# Autodesk Inventor assembly: independent_wheel_pair
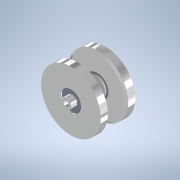
[picture p0: Inventor's stored thumbnail of the model, 180x180]
Saved by Autodesk Inventor 2020.3 (Build 243373000, 373)
## iProperties
Created: 2021-03-25
Part Number: independent_wheel_pair
Document SubType Name: Assembly
Designer: patry
Mass: 73.5609 g
Surface Area: 155.822 cm^2
Volume: 27.2448 cm^3
Density: 2.7 g/cm^3
Author: patry
## Documents named in this file (5)
- C:\Users\patry\Desktop\Konar staff\Ariadna2.1\ariadna_mechanika\Obszar roboczy\Naped\Zawieszenie_v3\independent_wheel_pair.iam
- C:\Users\patry\Desktop\Konar staff\Ariadna2.1\ariadna_mechanika\Obszar roboczy\Naped\Kola\single_wheel.iam
- C:\Users\patry\Desktop\Konar staff\Ariadna2.1\ariadna_mechanika\Obszar roboczy\Naped\Sruby\M5_nut_5mm.ipt
- C:\Users\patry\Desktop\Konar staff\Ariadna2.1\ariadna_mechanika\Obszar roboczy\Naped\Sruby\M5x35.ipt
- C:\Users\patry\Desktop\Konar staff\Ariadna2.1\ariadna_mechanika\Obszar roboczy\Naped\Sruby\M5_pad.ipt
## Components (7 placed, 4 different names)
1. single_wheel:1 [sub-assembly] — Zestawiające:1, Zestawiające:2, Zestawiające:6, Zestawiające:10
2. single_wheel:2 [sub-assembly] — Zestawiające:1, Zestawiające:2, Zestawiające:3, Zestawiające:4, Zestawiające:7
3. M5_nut_5mm:1 — Zestawiające:5, Zestawiające:6
4. M5x35:1 — Zestawiające:3, Zestawiające:4, Zestawiające:5, Zestawiające:8, Zestawiające:9, Zestawiające:11
5. M5_pad:1 — Zestawiające:7, Zestawiające:8
6. M5_nut_5mm:4 — Zestawiające:11, Zestawiające:12
7. M5_pad:2 — Zestawiające:9, Zestawiające:10, Zestawiające:12
## Relationships (12: Mate 12)
- Zestawiające:1 [Mate] (15 mm): single_wheel:1 ↔ single_wheel:2
- Zestawiające:2 [Mate]: single_wheel:1 ↔ single_wheel:2
- Zestawiające:3 [Mate]: single_wheel:2 ↔ M5x35:1
- Zestawiające:4 [Mate]: single_wheel:2 ↔ M5x35:1
- Zestawiające:5 [Mate]: M5_nut_5mm:1 ↔ M5x35:1
- Zestawiające:6 [Mate]: single_wheel:1 ↔ M5_nut_5mm:1
- Zestawiające:7 [Mate] (-0.25 mm): single_wheel:2 ↔ M5_pad:1
- Zestawiające:8 [Mate]: M5x35:1 ↔ M5_pad:1
- Zestawiające:9 [Mate]: M5x35:1 ↔ M5_pad:2
- Zestawiające:10 [Mate] (-0.25 mm): single_wheel:1 ↔ M5_pad:2
- Zestawiające:11 [Mate]: M5x35:1 ↔ M5_nut_5mm:4
- Zestawiające:12 [Mate] (4 mm): M5_nut_5mm:4 ↔ M5_pad:2
